# Autodesk Inventor assembly: 2AM-17-A-0200 - slider motor and gearbox
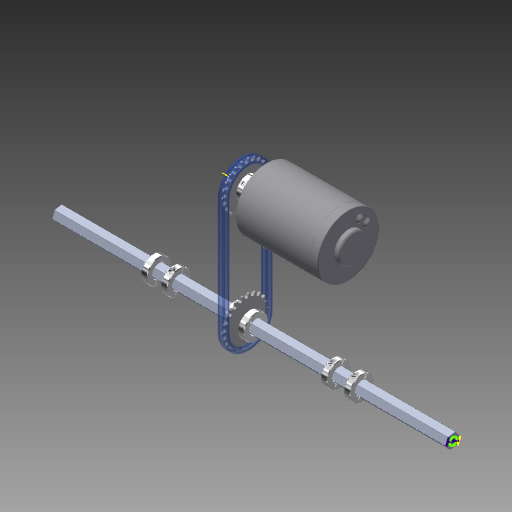
[picture p0: Inventor's stored thumbnail of the model, 512x512]
Saved by Autodesk Inventor 2017 (Build 210142000, 142)
## iProperties
Created: 2017-12-28
Part Number: 2AM-17-A-0200 - slider motor and gearbox
Document SubType Name: Assembly
Designer: Micah
Author: Micah
## Documents named in this file (8)
- C:\Users\Micah\Desktop\inventor\CADathon-2017\2AM-17-A-0200 - Smokestack Elevator\2AM-17-A-7200 - slider motor and gearbox.iam
- C:\Users\Micah\Desktop\inventor\CADathon-2017\2AM-17-A-0200 - Smokestack Elevator\COTS\217-3371-STEP.ipt
- C:\Users\Micah\Desktop\inventor\CADathon-2017\2AM-17-A-0200 - Smokestack Elevator\COTS\217-2761-STEP.ipt
- C:\Users\Micah\Desktop\inventor\CADathon-2017\2AM-17-A-0200 - Smokestack Elevator\COTS\217-3255-STEP.ipt
- C:\Users\Micah\Desktop\inventor\CADathon-2017\2AM-17-A-0200 - Smokestack Elevator\COTS\217-2737.20121205.ipt
- C:\Users\Micah\Desktop\inventor\CADathon-2017\2AM-17-A-0200 - Smokestack Elevator\2AM-17-P-7201 - sproket thing ig.ipt
- C:\Users\Micah\Desktop\inventor\CADathon-2017\2AM-17-A-0200 - Smokestack Elevator\2AM-17-A-7200 - slider motor and gearbox\Design Accelerator\Chain Drive2.iam
- C:\Users\Micah\Desktop\inventor\CADathon-2017\2AM-17-A-0200 - Smokestack Elevator\2AM-17-P-0204 - top hex shaft.ipt
## Components (14 placed, 7 different names)
1. 217-2761-STEP:2 — Mate:1
2. 217-3255-STEP:1 — Insert:1
3. 217-2737.20121205:1 — Rotational:2
4. 217-3371-STEP:1 — Mate:1, Insert:1, Rotational:2, Rotational:3, Rotational:4
5. 217-2737.20121205:2 — Rotational:3
6. 2AM-17-P-7201 - sproket thing ig:1 — Rotational:4
7. Chain Drive:1 [sub-assembly] — Rigid:9
8. 2AM-17-P-0204 - top hex shaft:1 — Rigid:9, Rigid:14, Rigid:15, Rigid:16, Rigid:17
9. 217-2737.20121205:3 — Rigid:15
10. 217-2737.20121205:4 — Rigid:14
11. 217-2737.20121205:6
12. 217-2737.20121205:8
13. 217-2737.20121205:9 — Rigid:17
14. 217-2737.20121205:10 — Rigid:16
## Relationships (10: WeldJoint 5, RevoluteJoint 3, Mate 1, Insert 1)
- Mate:1: 217-2761-STEP:2 ↔ 217-3371-STEP:1
- Insert:1 (-28.575 mm): 217-3255-STEP:1 ↔ 217-3371-STEP:1
- Rotational:2 [RevoluteJoint] (-11.43 mm): 217-2737.20121205:1 ↔ 217-3371-STEP:1
- Rotational:3 [RevoluteJoint] (-16.51 mm): 217-3371-STEP:1 ↔ 217-2737.20121205:2
- Rotational:4 [RevoluteJoint] (-15.24 mm): 217-3371-STEP:1 ↔ 2AM-17-P-7201 - sproket thing ig:1
- Rigid:9 [WeldJoint] (-215.9 mm): Chain Drive:1 ↔ 2AM-17-P-0204 - top hex shaft:1
- Rigid:14 [WeldJoint] (-309.5625 mm): 2AM-17-P-0204 - top hex shaft:1 ↔ 217-2737.20121205:4
- Rigid:15 [WeldJoint] (-282.575 mm): 2AM-17-P-0204 - top hex shaft:1 ↔ 217-2737.20121205:3
- Rigid:16 [WeldJoint] (-117.475 mm): 2AM-17-P-0204 - top hex shaft:1 ↔ 217-2737.20121205:10
- Rigid:17 [WeldJoint] (-93.6625 mm): 2AM-17-P-0204 - top hex shaft:1 ↔ 217-2737.20121205:9
